# Autodesk Inventor assembly: ASY PRS 2 Filter column D1200 940
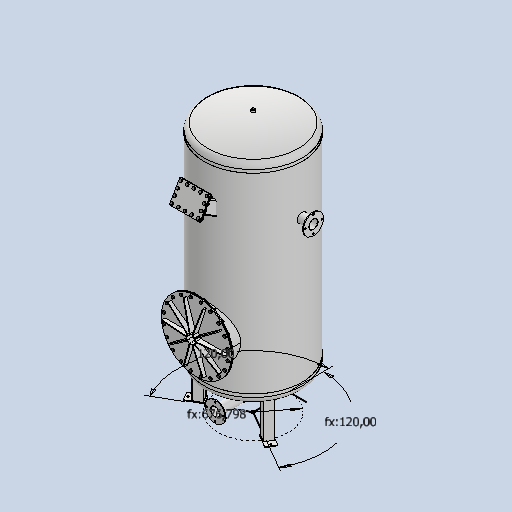
[picture p0: Inventor's stored thumbnail of the model, 512x512]
Saved by Autodesk Inventor 2026.2 (Build 302298010, 298A)
## iProperties
Created: 2025-02-13
Part Number: ASY PRS 2 Filter column D1200 940
Document SubType Name: Assembly
Designer: admin
Mass: 296006 g
Surface Area: 199460 cm^2
Volume: 66339.5 cm^3
Density: 4.46198 g/cm^3
Author: pokla
Revision Number: 3
## Documents named in this file (11)
- C:\Users\admin\Documents\Inventor\PRS-Purovsk\ASY PRS 2 Filter column D1200 940.iam
- C:\Users\admin\Documents\Inventor\PRS-Purovsk\PRS 0101 main shell D1200.ipt
- C:\Users\admin\Documents\Inventor\PRS-Purovsk\PRS 0101 main shell D1200 940.ipt
- C:\Users\admin\Documents\Inventor\PRS-Purovsk\PRS 1604 dished head_D1200 940.ipt
- C:\Users\admin\Documents\Inventor\PRS-Purovsk\Fitting G1_D1200 940.ipt
- C:\Users\admin\Documents\Inventor\PRS-Purovsk\PRS 8123 pallet jack dummy_D1200.ipt
- C:\Users\admin\Documents\Inventor\PRS-Purovsk\ASY PRS 9690 Filter legs D1200 940.iam
- C:\Users\admin\Documents\Inventor\PRS-Purovsk\ASY PRS 9600 charging hatch.iam
- C:\Users\admin\Documents\Inventor\PRS-Purovsk\ASY PRS 9500 inlet pipe.iam
- C:\Users\admin\Documents\Inventor\PRS-Purovsk\ASY PRS 9600 accses hatch.iam
- C:\Users\admin\Documents\Inventor\PRS-Purovsk\ASY PRS 9700 outlet pipe.iam
## Components (11 placed, 9 different names)
1. PRS 0101 main shell D1200 940:1 — Mate:1, Flush:4, Flush:2, Rotational:2, Rotational:3
2. PRS 1604 dished head_D1200 940:1 — Mate:8, Mate:5, Mate:147, Mate:148, Rotational:2
3. PRS 1604 dished head_D1200 940:2 — Rigid:15, Rotational:3
4. Fitting G1_D1200 940:1 — Rigid:15
5. PRS 8123 pallet jack dummy_D1200:1
6. Fitting G1_D1200 940:2 — Mate:8, Mate:7, Mate:6
7. ASY PRS 9690 Filter legs D1200 940:1 [sub-assembly] — Mate:2, Flush:6, Flush:5
8. ASY PRS 9600 charging hatch:1 [sub-assembly]
9. ASY PRS 9500 inlet pipe:1 [sub-assembly]
10. ASY PRS 9600 accses hatch:1 [sub-assembly]
11. ASY PRS 9700 outlet pipe:1 [sub-assembly]
## Relationships (20: Mate 11, Flush 4, WeldJoint 3, RevoluteJoint 2)
- Mate:1: PRS 0101 main shell D1200 940:1
- Flush:4: PRS 0101 main shell D1200 940:1
- Flush:2: PRS 0101 main shell D1200 940:1
- [Mate]: PRS 0101 main shell D1200 940:1 ↔ ASY PRS 9600 charging hatch:1
- [Mate]: PRS 0101 main shell D1200 940:1 ↔ ASY PRS 9600 charging hatch:1
- [Mate]: PRS 1604 dished head_D1200 940:2 ↔ ASY PRS 9500 inlet pipe:1
- Mate:8: PRS 1604 dished head_D1200 940:1 ↔ Fitting G1_D1200 940:2
- Mate:7 (150 mm): Fitting G1_D1200 940:2
- Mate:6: Fitting G1_D1200 940:2
- Mate:2: ASY PRS 9690 Filter legs D1200 940:1
- Flush:6: ASY PRS 9690 Filter legs D1200 940:1
- Flush:5: ASY PRS 9690 Filter legs D1200 940:1
- Rigid:15 [WeldJoint]: PRS 1604 dished head_D1200 940:2 ↔ Fitting G1_D1200 940:1
- [WeldJoint] (20 mm): PRS 0101 main shell D1200 940:1 ↔ ASY PRS 9600 accses hatch:1
- [WeldJoint]: PRS 1604 dished head_D1200 940:1 ↔ ASY PRS 9700 outlet pipe:1
- Mate:5 (300 mm): PRS 1604 dished head_D1200 940:1
- Mate:147: PRS 1604 dished head_D1200 940:1
- Mate:148: PRS 1604 dished head_D1200 940:1
- Rotational:2 [RevoluteJoint]: PRS 0101 main shell D1200 940:1 ↔ PRS 1604 dished head_D1200 940:1
- Rotational:3 [RevoluteJoint]: PRS 0101 main shell D1200 940:1 ↔ PRS 1604 dished head_D1200 940:2
## Named parameters: AA_MAIN_filter_diam = 1200 mm, AccsessHatch_tube_diameter = 530 mm, ChargingHatch_width = 208 mm, ChargingHatch_hight = 122 mm, AA_MAIN_Filter_Clearance = 300 mm, Legs_Tube_lenght = 417.45004 mm, Legs_Tube_cut_angle = 0.41416, Legs_Upper_plate_lenght = 122.38827 mm, Legs_Tube_dim = 80 mm, Legs_Inner_diam = 895.69544 mm
note: some values were not read from the file. Shown as the stored number, unit unknown: "Legs_Tube_cut_angle".
